# Autodesk Inventor assembly: ensamble
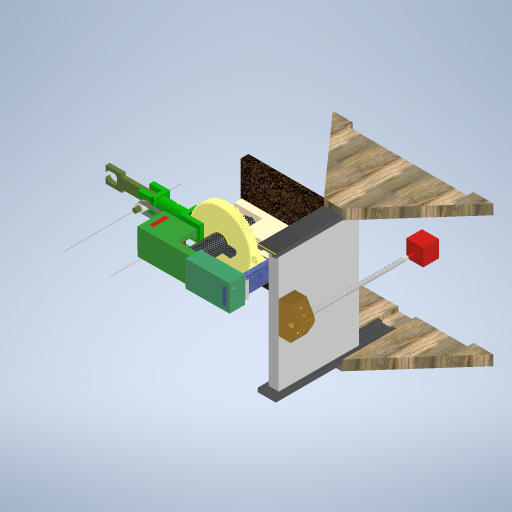
[picture p0: Inventor's stored thumbnail of the model, 512x512]
Saved by Autodesk Inventor 2023 (Build 270158000, 158)
## iProperties
Created: 2024-07-31
Part Number: ensamble
Document SubType Name: Assembly
Designer: sebas
Author: sebas
## Documents named in this file (21)
- E:\Unlz\PROYECTO FINAL\recibida\ensamble.iam
- E:\Unlz\PROYECTO FINAL\recibida\base.ipt
- E:\Unlz\PROYECTO FINAL\recibida\techo.ipt
- E:\Unlz\PROYECTO FINAL\recibida\eje.ipt
- E:\Unlz\PROYECTO FINAL\recibida\pared.ipt
- E:\Unlz\PROYECTO FINAL\recibida\techo2.ipt
- E:\Unlz\PROYECTO FINAL\recibida\engranje.ipt
- E:\Unlz\PROYECTO FINAL\recibida\braazo1.ipt
- E:\Unlz\PROYECTO FINAL\recibida\brazo2.ipt
- E:\Unlz\PROYECTO FINAL\recibida\motor.ipt
- E:\Unlz\PROYECTO FINAL\recibida\engranaje2.iam.ipt
- E:\Unlz\PROYECTO FINAL\recibida\TENSOR.ipt
- E:\Unlz\PROYECTO FINAL\recibida\Part1.0002.ipt
- E:\Unlz\PROYECTO FINAL\recibida\GUIA INTERIOR.0003.ipt
- E:\Unlz\PROYECTO FINAL\recibida\base vertical.0002.ipt
- E:\Unlz\PROYECTO FINAL\recibida\base horiz.0004.ipt
- E:\Unlz\PROYECTO FINAL\recibida\escuadra.0001.ipt
- E:\Unlz\PROYECTO FINAL\recibida\sin fin.0002.ipt
- E:\Unlz\PROYECTO FINAL\recibida\encatre sin fin.0002.ipt
- E:\Unlz\PROYECTO FINAL\recibida\ensamble\Design Accelerator\Synchronous Belts Transmission2.iam
- engranaje2.iam
## Components (23 placed, 19 different names)
1. base:1 — Mate:10, Mate:22, Mate:23, Mate:24, Mate:25, Mate:28, Flush:24, Mate:31, Mate:32, Mate:47, Mate:48, Flush:36, Symmetry:2
2. techo:1 — Mate:7, Mate:8, Mate:9, Mate:30, Mate:33, Mate:34, Flush:26, Mate:38, Flush:27, Mate:39, Symmetry:1, Mate:56, Flush:42, Flush:43, Mate:57
3. eje:1 — Mate:23, Mate:24, Mate:29, Mate:30
4. pared:1 — Flush:24, Mate:31, Mate:32, Flush:25, Symmetry:2
5. techo2:2 — Mate:7, Mate:8, Mate:9, Flush:25, Symmetry:1
6. engranje:1 — Mate:10, Flush:22, Mate:19, Flush:23, Mate:22, Mate:29
7. braazo1:1 — Flush:22, Mate:19, Flush:23, Mate:20, Mate:21, Symmetry:3, Flush:43
8. brazo2:1 — Mate:20, Mate:21, Symmetry:3, Mate:57
9. motor:3 — Mate:33, Mate:34, Flush:26
10. engranaje2.iam:1
11. TENSOR:1 — Mate:38, Flush:27, Mate:39
12. Part1.0002:1 — Mate:45, Mate:46, Flush:37, Mate:51, Mate:52, Flush:40
13. Part1.0002:2 — Mate:42, Mate:43, Flush:37, Mate:49, Mate:50
14. GUIA INTERIOR.0003:1 — Mate:41, Flush:30, Flush:31, Mate:42, Mate:43
15. GUIA INTERIOR.0003:2 — Mate:44, Flush:32, Flush:33, Mate:45, Mate:46
16. base vertical.0002:1 — Mate:40, Flush:28, Flush:29, Mate:41, Flush:30, Flush:31, Mate:44, Flush:32, Flush:33, Mate:48, Mate:54, Flush:39
17. base horiz.0004:1 — Mate:40, Flush:28, Flush:29, Mate:47, Flush:36
18. escuadra.0001:1 — Mate:49, Mate:50, Flush:38
19. escuadra.0001:2 — Mate:51, Mate:52, Flush:38, Flush:41
20. sin fin.0002:1 — Insert:1, Mate:55
21. encatre sin fin.0002:1 — Mate:54, Flush:39, Flush:40, Insert:1
22. motor:4 — Mate:55, Flush:41
23. Synchronous Belts Transmission:1 [sub-assembly]
## Relationships (61: Mate 37, Flush 20, Symmetry 3, Insert 1)
- Mate:7: techo:1 ↔ techo2:2
- Mate:8: techo:1 ↔ techo2:2
- Mate:9: techo:1 ↔ techo2:2
- Mate:10: base:1 ↔ engranje:1
- Flush:22: engranje:1 ↔ braazo1:1
- Mate:19 (0.25 mm): engranje:1 ↔ braazo1:1
- Flush:23: engranje:1 ↔ braazo1:1
- Mate:20: braazo1:1 ↔ brazo2:1
- Mate:21 (4 mm): braazo1:1 ↔ brazo2:1
- Mate:22 (2 mm): base:1 ↔ engranje:1
- Mate:23: base:1 ↔ eje:1
- Mate:24: base:1 ↔ eje:1
- Mate:25: base:1
- Mate:28: base:1
- Mate:29 (0.3 mm): eje:1 ↔ engranje:1
- Mate:30: techo:1 ↔ eje:1
- Flush:24: base:1 ↔ pared:1
- Mate:31 (0.3 mm): base:1 ↔ pared:1
- Mate:32 (0.25 mm): base:1 ↔ pared:1
- Flush:25: pared:1 ↔ techo2:2
- Mate:33: techo:1 ↔ motor:3
- Mate:34: techo:1 ↔ motor:3
- Flush:26: techo:1 ↔ motor:3
- Mate:38: techo:1 ↔ TENSOR:1
- Flush:27: techo:1 ↔ TENSOR:1
- Mate:39: techo:1 ↔ TENSOR:1
- Mate:40: base vertical.0002:1 ↔ base horiz.0004:1
- Flush:28 (-25 mm): base vertical.0002:1 ↔ base horiz.0004:1
- Flush:29: base vertical.0002:1 ↔ base horiz.0004:1
- Mate:41: GUIA INTERIOR.0003:1 ↔ base vertical.0002:1
- Flush:30: GUIA INTERIOR.0003:1 ↔ base vertical.0002:1
- Flush:31: GUIA INTERIOR.0003:1 ↔ base vertical.0002:1
- Mate:42: Part1.0002:2 ↔ GUIA INTERIOR.0003:1
- Mate:43: Part1.0002:2 ↔ GUIA INTERIOR.0003:1
- Mate:44: GUIA INTERIOR.0003:2 ↔ base vertical.0002:1
- Flush:32: GUIA INTERIOR.0003:2 ↔ base vertical.0002:1
- Flush:33: GUIA INTERIOR.0003:2 ↔ base vertical.0002:1
- Mate:45: Part1.0002:1 ↔ GUIA INTERIOR.0003:2
- Mate:46: Part1.0002:1 ↔ GUIA INTERIOR.0003:2
- Mate:47: base:1 ↔ base horiz.0004:1
- Mate:48 (70 mm): base:1 ↔ base vertical.0002:1
- Flush:36 (100 mm): base:1 ↔ base horiz.0004:1
- Flush:37: Part1.0002:1 ↔ Part1.0002:2
- Mate:49: Part1.0002:2 ↔ escuadra.0001:1
- Mate:50: Part1.0002:2 ↔ escuadra.0001:1
- Mate:51: Part1.0002:1 ↔ escuadra.0001:2
- Mate:52: Part1.0002:1 ↔ escuadra.0001:2
- Flush:38: escuadra.0001:1 ↔ escuadra.0001:2
- Mate:54: base vertical.0002:1 ↔ encatre sin fin.0002:1
- Flush:39: base vertical.0002:1 ↔ encatre sin fin.0002:1
- Flush:40 (130 mm): Part1.0002:1 ↔ encatre sin fin.0002:1
- Insert:1: sin fin.0002:1 ↔ encatre sin fin.0002:1
- Mate:55: sin fin.0002:1 ↔ motor:4
- Flush:41: escuadra.0001:2 ↔ motor:4
- Symmetry:1: techo:1 ↔ techo2:2
- Mate:56: techo:1
- Symmetry:2: base:1 ↔ pared:1
- Flush:42: techo:1
- Symmetry:3: braazo1:1 ↔ brazo2:1
- Flush:43: techo:1 ↔ braazo1:1
- Mate:57: techo:1 ↔ brazo2:1
